# Autodesk Inventor assembly: 22-130
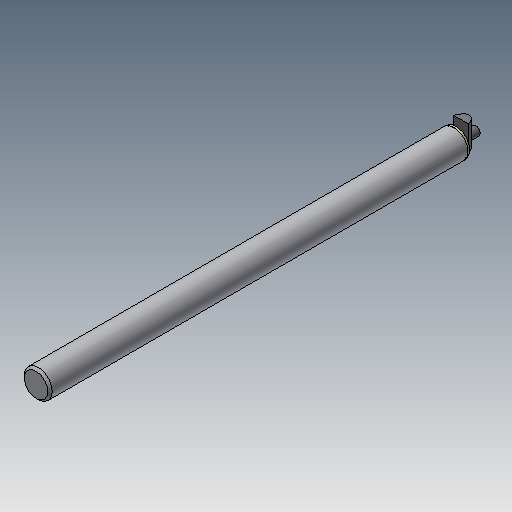
[picture p0: Inventor's stored thumbnail of the model, 512x512]
Saved by Autodesk Inventor 2018.3 (Build 223284000, 284)
## iProperties
Created: 2004-11-24
Part Number: 22-130
Document SubType Name: Assembly
Designer: Autodesk, Inc.
Manufacturer: Standard
Standards Organization: Custom
Description: BIN MOUNTING SLIDE RAIL
Vendor: PARKER IPS
Catalog Web Link: http://www.parker.com/ead/cm1.asp?cmid=809
Mass: 535.837 g
Surface Area: 338.387 cm^2
Volume: 195.64 cm^3
Density: 2.73889 g/cm^3
CAGE: 1LJX3
Dept. ID: Product Design
Description #2: ---
Finish #1: ---
Finish #2: ---
Material ID: ---
Project Number: ---
Author: Autodesk, Inc.
## Documents named in this file (5)
- C:\AVAInvAPI\Workspace\Test Station\Components\22-130.iam
- C:\AVAInvAPI\Workspace\Test Station\Components\22-130.ipt
- C:\AVAInvAPI\Workspace\Test Station\Components\20-058.ipt
- C:\AVAInvAPI\Workspace\Test Station\Components\Nylon Washer.ipt
- C:\Users\kelleyb.ADS\Desktop\Samples MIGRATED 2009 224 RTM_1\Standard Parts\Test Station Content\Fastners\20-XXX TSlot Nuts.ipt
## Components (3 placed, 3 different names)
1. 22-130:1 — Mate:1, Flush:1
2. 20-058:1 — Mate:1, Mate:2
3. Nylon Washer:1 — Flush:1, Mate:2
## Relationships (3: Mate 2, Flush 1)
- Mate:1: 22-130:1 ↔ 20-058:1
- Flush:1: 22-130:1 ↔ Nylon Washer:1
- Mate:2 (4.5 mm): 20-058:1 ↔ Nylon Washer:1
